# Autodesk Inventor assembly: thumbL2
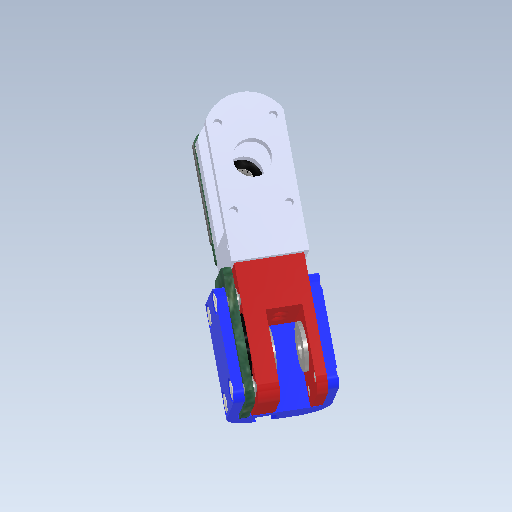
[picture p0: Inventor's stored thumbnail of the model, 512x512]
Saved by Autodesk Inventor 2020 (Build 240168000, 168)
## iProperties
Created: 2020-04-30
Part Number: thumbL2
Document SubType Name: Assembly
Designer: sami_
Author: sami_
## Documents named in this file (11)
- C:\Users\sami_\Documents\V1.6\thumbL2.iam
- C:\Users\sami_\Documents\V1.6\Libraries\Content Center Files\en-US\ISO 7089\ISO 7089 - 1.6 - 140 HV(1).ipt
- C:\Users\sami_\Documents\V1.6\Libraries\Content Center Files\en-US\ISO 1224-1 M\ISO 1224-1 - 17 - 4 x 7 x 2.ipt
- C:\Users\sami_\Documents\V1.6\Libraries\Content Center Files\en-US\ISO 7089\ISO 7089 - 4 - 140 HV(1).ipt
- C:\Users\sami_\Documents\V1.6\Workgroups\NotInProject\THUMB\Assembly\PotentiometerAssembly.iam
- C:\Users\sami_\Documents\V1.6\Workgroups\NotInProject\THUMB\Assembly\New Thumb with Correct joint 2.0.ipt
- C:\Users\sami_\Documents\V1.6\Workgroups\NotInProject\fingerpanel.ipt
- C:\Users\sami_\Documents\Inventor\Content Center Files\R2020\en-US\AS 1427(03)\AS 1427 - M2 x 8(1).ipt
- C:\Users\sami_\Documents\Inventor\Content Center Files\R2020\en-US\AS 1427(03)\AS 1427 - M2 x 4(1).ipt
- C:\Users\sami_\Documents\V1.6\Workgroups\NotInProject\THUMB\nonpcbback.ipt
- C:\Users\sami_\Documents\Inventor\Content Center Files\R2020\en-US\AS 1427(03)\AS 1427 - M2 x 6(1).ipt
## Components (29 placed, 10 different names)
1. ISO 7089 1.6:1
2. ISO 7089 1.6:2
3. ISO 7089 1.6:3
4. ISO 7089 1.6:4
5. ISO 1224-1 (Metric) 17 - 4 x 7 x 2:1
6. ISO 1224-1 (Metric) 17 - 4 x 7 x 2:2
7. ISO 7089 4:1
8. ISO 7089 4:2
9. PotentiometerAssembly:1 [sub-assembly]
10. PotentiometerAssembly:2 [sub-assembly] — Rigid:18, Rigid:19
11. New Thumb with Correct joint 2.0:1 — Rigid:19
12. ISO 7089 1.6:5
13. ISO 7089 1.6:6
14. ISO 7089 1.6:7
15. ISO 7089 1.6:8
16. fingerpanel:1 — Mate:8, Mate:9, Mate:10, Mate:11, Mate:12, Mate:13, Mate:14, Mate:15
17. AS 1427 - Metric M2 x 8:1 — Mate:8
18. AS 1427 - Metric M2 x 8:2 — Mate:9
19. AS 1427 - Metric M2 x 8:3 — Mate:10
20. AS 1427 - Metric M2 x 8:4 — Mate:11
21. AS 1427 - Metric M2 x 4:4 — Mate:12
22. AS 1427 - Metric M2 x 4:1 — Mate:13
23. AS 1427 - Metric M2 x 4:2 — Mate:14
24. AS 1427 - Metric M2 x 4:3 — Mate:15
25. nonpcbback:1 — Rigid:18, Mate:16, Mate:17, Mate:18, Mate:19
26. AS 1427 - Metric M2 x 6:1 — Mate:16
27. AS 1427 - Metric M2 x 6:2 — Mate:17
28. AS 1427 - Metric M2 x 6:3 — Mate:18
29. AS 1427 - Metric M2 x 6:4 — Mate:19
## Relationships (28: WeldJoint 15, Mate 13)
- [WeldJoint]: ISO 7089 1.6:4 ↔ PotentiometerAssembly:1
- [WeldJoint]: ISO 7089 1.6:3 ↔ PotentiometerAssembly:1
- [WeldJoint]: ISO 7089 1.6:1 ↔ PotentiometerAssembly:1
- [WeldJoint]: ISO 7089 1.6:2 ↔ PotentiometerAssembly:1
- [WeldJoint]: ISO 1224-1 (Metric) 17 - 4 x 7 x 2:1 ↔ ISO 7089 4:1
- [WeldJoint]: ISO 7089 4:1 ↔ New Thumb with Correct joint 2.0:1
- [WeldJoint]: PotentiometerAssembly:2 ↔ ISO 7089 1.6:8
- [WeldJoint]: PotentiometerAssembly:2 ↔ ISO 7089 1.6:5
- [WeldJoint]: PotentiometerAssembly:2 ↔ ISO 7089 1.6:6
- [WeldJoint]: PotentiometerAssembly:2 ↔ ISO 7089 1.6:7
- [Mate] (0.3 mm): ISO 7089 1.6:3 ↔ New Thumb with Correct joint 2.0:1
- [WeldJoint]: ISO 1224-1 (Metric) 17 - 4 x 7 x 2:2 ↔ ISO 7089 4:2
- [WeldJoint]: ISO 7089 4:2 ↔ New Thumb with Correct joint 2.0:1
- [WeldJoint]: New Thumb with Correct joint 2.0:1 ↔ fingerpanel:1
- Mate:8: fingerpanel:1 ↔ AS 1427 - Metric M2 x 8:1
- Mate:9: fingerpanel:1 ↔ AS 1427 - Metric M2 x 8:2
- Mate:10: fingerpanel:1 ↔ AS 1427 - Metric M2 x 8:3
- Mate:11: fingerpanel:1 ↔ AS 1427 - Metric M2 x 8:4
- Mate:12: fingerpanel:1 ↔ AS 1427 - Metric M2 x 4:4
- Mate:13: fingerpanel:1 ↔ AS 1427 - Metric M2 x 4:1
- Mate:14: fingerpanel:1 ↔ AS 1427 - Metric M2 x 4:2
- Mate:15: fingerpanel:1 ↔ AS 1427 - Metric M2 x 4:3
- Rigid:18 [WeldJoint]: PotentiometerAssembly:2 ↔ nonpcbback:1
- Rigid:19 [WeldJoint] (0.5 mm): PotentiometerAssembly:2 ↔ New Thumb with Correct joint 2.0:1
- Mate:16: nonpcbback:1 ↔ AS 1427 - Metric M2 x 6:1
- Mate:17: nonpcbback:1 ↔ AS 1427 - Metric M2 x 6:2
- Mate:18: nonpcbback:1 ↔ AS 1427 - Metric M2 x 6:3
- Mate:19: nonpcbback:1 ↔ AS 1427 - Metric M2 x 6:4
